# Autodesk Inventor assembly: 203.001.01_ZB_Modul
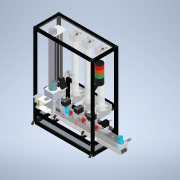
[picture p0: Inventor's stored thumbnail of the model, 180x180]
Saved by Autodesk Inventor 2022 (Build 260153000, 153)
## iProperties
Created: 2021-12-04
Part Number: 203.001.01_ZB_Modul
Document SubType Name: Assembly
Designer: Sebastian Seewald
Author: Sebastian Seewald
## Documents named in this file (18)
- C:\Users\kaebi\OneDrive - mci4me.at\03_MCI Master\4.Semester_SS2022\Masterarbeit\Software\CAD_TeachingFactory\203.001.01_ZB_Modul.iam
- C:\Users\kaebi\OneDrive - mci4me.at\03_MCI Master\4.Semester_SS2022\Masterarbeit\Software\CAD_TeachingFactory\202.002.01_ZB_Rahmen_Modul.iam
- C:\Users\kaebi\OneDrive - mci4me.at\03_MCI Master\4.Semester_SS2022\Masterarbeit\Software\CAD_TeachingFactory\503.001.01_Statuslampe.ipt
- C:\Users\kaebi\OneDrive - mci4me.at\03_MCI Master\4.Semester_SS2022\Masterarbeit\Software\CAD_TeachingFactory\DIN 934 - M4 x 0.7 Mutter.ipt
- C:\Users\kaebi\OneDrive - mci4me.at\03_MCI Master\4.Semester_SS2022\Masterarbeit\Software\CAD_TeachingFactory\204.006.01_ZB_Extrudereinheit.iam
- C:\Users\kaebi\OneDrive - mci4me.at\03_MCI Master\4.Semester_SS2022\Masterarbeit\Software\CAD_TeachingFactory\DIN 6902 - M4 Unterlegscheibe.ipt
- C:\Users\kaebi\OneDrive - mci4me.at\03_MCI Master\4.Semester_SS2022\Masterarbeit\Software\CAD_TeachingFactory\DIN 912 - M4 x 20.ipt
- C:\Users\kaebi\OneDrive - mci4me.at\03_MCI Master\4.Semester_SS2022\Masterarbeit\Software\CAD_TeachingFactory\204.005.01_ZB_Hubmagnetstopper.iam
- C:\Users\kaebi\OneDrive - mci4me.at\03_MCI Master\4.Semester_SS2022\Masterarbeit\Software\CAD_TeachingFactory\DIN EN ISO 4762 - M4 x 10.ipt
- C:\Users\kaebi\OneDrive - mci4me.at\03_MCI Master\4.Semester_SS2022\Masterarbeit\Software\CAD_TeachingFactory\205.001.01_ZB_Foerderbandeinheit.iam
- C:\Users\kaebi\OneDrive - mci4me.at\03_MCI Master\4.Semester_SS2022\Masterarbeit\Software\CAD_TeachingFactory\DIN_912_M3x8.ipt
- C:\Users\kaebi\OneDrive - mci4me.at\03_MCI Master\4.Semester_SS2022\Masterarbeit\Software\CAD_TeachingFactory\206.001.01_Vereinzelung_Gesamtbaugruppe.iam
- 206.001.01_Vereinzelung_Gesamtbaugruppe.iam
- C:\Users\kaebi\OneDrive - mci4me.at\03_MCI Master\4.Semester_SS2022\Masterarbeit\Software\CAD_TeachingFactory\503.002.01_Laborflaschen.ipt
- C:\Users\kaebi\OneDrive - mci4me.at\03_MCI Master\4.Semester_SS2022\Masterarbeit\Software\CAD_TeachingFactory\506.007.01_Linearaktor.iam
- C:\Users\kaebi\OneDrive - mci4me.at\03_MCI Master\4.Semester_SS2022\Masterarbeit\Software\CAD_TeachingFactory\106.023.01_Zapfen_Aktor.ipt
- C:\Users\kaebi\OneDrive - mci4me.at\03_MCI Master\4.Semester_SS2022\Masterarbeit\Software\CAD_TeachingFactory\106.024.01_Zapfen_Aktor_Auflage.ipt
- C:\Users\kaebi\OneDrive - mci4me.at\03_MCI Master\4.Semester_SS2022\Masterarbeit\Software\CAD_TeachingFactory\106.025.01_Anbindung_Aktor.ipt
## Components (70 placed, 16 different names)
1. 202.002.01_ZB_Rahmen_Modul:1 [sub-assembly] — Passend:1, Passend:2, Passend:3, Passend:6, Passend:7, Passend:8, Passend:9, Passend:10, Passend:11, Passend:12, Passend:13, Passend:14, Passend:15, Passend:16, Passend:17, Passend:18, Passend:19, Passend:20, Passend:21, Passend:22, Passend:23, Passend:24, Passend:25, Passend:26, Passend:27, Passend:28, Passend:65, Passend:66, Passend:67, Passend:68, Passend:69, Winkel:1, Winkel:2, Winkel:3, Passend:95, Fluchtend:1, Passend:96, Passend:121, Fluchtend:2, Passend:122, Passend:129, Passend:146, Fluchtend:5, Passend:147
2. 503.001.01_Statuslampe:1 — Passend:1, Passend:2, Passend:3, Passend:4, Passend:5
3. DIN 934 - M4 x 0.7 Mutter:1 — Passend:4, Passend:6
4. DIN 934 - M4 x 0.7 Mutter:2 — Passend:5, Passend:7
5. 204.006.01_ZB_Extrudereinheit:1 [sub-assembly] — Passend:8, Passend:13, Passend:14, Passend:29, Passend:30, Passend:31, Passend:32, Passend:97, Passend:98, Passend:128
6. 204.006.01_ZB_Extrudereinheit:2 [sub-assembly] — Passend:9, Passend:12, Passend:15, Passend:33, Passend:34, Passend:35, Passend:36, Passend:99, Passend:100, Passend:127
7. 204.006.01_ZB_Extrudereinheit:3 [sub-assembly] — Passend:10, Passend:11, Passend:16, Passend:37, Passend:38, Passend:39, Passend:40, Passend:101, Passend:102, Passend:124, Fluchtend:3
8. DIN 6902 - M4 Unterlegscheibe:1 — Passend:20, Passend:37, Passend:43, Passend:55
9. DIN 6902 - M4 Unterlegscheibe:2 — Passend:18, Passend:39, Passend:41, Passend:53
10. DIN 6902 - M4 Unterlegscheibe:3 — Passend:17, Passend:40, Passend:42, Passend:54
11. DIN 6902 - M4 Unterlegscheibe:4 — Passend:19, Passend:38, Passend:44, Passend:56
12. DIN 6902 - M4 Unterlegscheibe:5 — Passend:21, Passend:36, Passend:46, Passend:58
13. DIN 6902 - M4 Unterlegscheibe:6 — Passend:23, Passend:34, Passend:48, Passend:60
14. DIN 6902 - M4 Unterlegscheibe:7 — Passend:22, Passend:35, Passend:45, Passend:57
15. DIN 6902 - M4 Unterlegscheibe:8 — Passend:25, Passend:30, Passend:52, Passend:63
16. DIN 6902 - M4 Unterlegscheibe:9 — Passend:26, Passend:31, Passend:51, Passend:61
17. DIN 6902 - M4 Unterlegscheibe:10 — Passend:24, Passend:33, Passend:47, Passend:59
18. DIN 6902 - M4 Unterlegscheibe:11 — Passend:28, Passend:29, Passend:50, Passend:64
19. DIN 6902 - M4 Unterlegscheibe:12 — Passend:27, Passend:32, Passend:49, Passend:62
20. DIN 912 - M4 x 20:1 — Passend:41, Passend:53
21. DIN 912 - M4 x 20:2 — Passend:44, Passend:56
22. DIN 912 - M4 x 20:3 — Passend:48, Passend:60
23. DIN 912 - M4 x 20:4 — Passend:51, Passend:61
24. DIN 912 - M4 x 20:5 — Passend:52, Passend:63
25. DIN 912 - M4 x 20:6 — Passend:47, Passend:59
26. DIN 912 - M4 x 20:7 — Passend:46, Passend:58
27. DIN 912 - M4 x 20:8 — Passend:43, Passend:55
28. DIN 912 - M4 x 20:9 — Passend:42, Passend:54
29. DIN 912 - M4 x 20:10 — Passend:45, Passend:57
30. DIN 912 - M4 x 20:11 — Passend:49, Passend:62
31. DIN 912 - M4 x 20:12 — Passend:50, Passend:64
32. 204.005.01_ZB_Hubmagnetstopper:1 [sub-assembly] — Passend:66, Passend:69, Winkel:2, Passend:76, Passend:77, Passend:78, Passend:79, Passend:85, Passend:86, Passend:91, Passend:92, Passend:127
33. 204.005.01_ZB_Hubmagnetstopper:2 [sub-assembly] — Passend:65, Winkel:1, Passend:80, Passend:81, Passend:82, Passend:83, Passend:87, Passend:88, Passend:89, Passend:90, Fluchtend:3
34. 204.005.01_ZB_Hubmagnetstopper:3 [sub-assembly] — Passend:67, Passend:68, Winkel:3, Passend:71, Passend:72, Passend:73, Passend:74, Passend:75, Passend:84, Passend:93, Passend:94, Passend:128
35. DIN EN ISO 4762 - M4 x 10:1 — Passend:71, Passend:72
36. DIN EN ISO 4762 - M4 x 10:2 — Passend:75, Passend:93
37. DIN EN ISO 4762 - M4 x 10:3 — Passend:74, Passend:94
38. DIN EN ISO 4762 - M4 x 10:4 — Passend:73, Passend:84
39. DIN EN ISO 4762 - M4 x 10:5 — Passend:76, Passend:85
40. DIN EN ISO 4762 - M4 x 10:6 — Passend:77, Passend:92
41. DIN EN ISO 4762 - M4 x 10:7 — Passend:78, Passend:86
42. DIN EN ISO 4762 - M4 x 10:8 — Passend:79, Passend:91
43. DIN EN ISO 4762 - M4 x 10:9 — Passend:82, Passend:90
44. DIN EN ISO 4762 - M4 x 10:10 — Passend:83, Passend:89
45. DIN EN ISO 4762 - M4 x 10:11 — Passend:81, Passend:88
46. DIN EN ISO 4762 - M4 x 10:12 — Passend:80, Passend:87, Passend:129
47. 205.001.01_ZB_Foerderbandeinheit:1 [sub-assembly] — Passend:95, Fluchtend:1, Passend:96, Passend:103, Passend:104, Passend:105, Passend:106, Passend:107, Passend:108, Passend:115, Passend:116, Passend:117, Passend:118, Passend:119, Passend:120, Passend:123, Passend:125, Passend:130, Passend:131
48. DIN_912_M3x8:1 — Passend:97, Passend:103, Passend:109
49. DIN_912_M3x8:2 — Passend:98, Passend:104, Passend:110
50. DIN_912_M3x8:3 — Passend:99, Passend:105, Passend:111
51. DIN_912_M3x8:4 — Passend:100, Passend:106, Passend:112
52. DIN_912_M3x8:5 — Passend:102, Passend:108, Passend:114
53. DIN_912_M3x8:6 — Passend:101, Passend:107, Passend:113
54. DIN_912_M3x8:7 — Passend:110, Passend:119
55. DIN_912_M3x8:8 — Passend:109, Passend:120
56. DIN_912_M3x8:9 — Passend:112, Passend:117
57. DIN_912_M3x8:10 — Passend:111, Passend:118
58. DIN_912_M3x8:11 — Passend:113, Passend:116
59. DIN_912_M3x8:12 — Passend:114, Passend:115
60. 206.001.01_Vereinzelung_Gesamtbaugruppe:1 [sub-assembly] — Passend:121, Fluchtend:2, Passend:122, Passend:148, Passend:149
61. 503.002.01_Laborflaschen:1 — Passend:123, Passend:124, Passend:125
62. 503.002.01_Laborflaschen:2 — Passend:130, Passend:131
63. 506.007.01_Linearaktor:1 [sub-assembly] — Passend:148
64. 102.004.01_Zapfen_Aktor:1
65. 102.004.01_Zapfen_Aktor:2
66. 102.005.01_Zapfen_Aktor_Auflage:1
67. 102.005.01_Zapfen_Aktor_Auflage:2
68. 106.025.01_Anbindung_Aktor:1
69. 106.025.01_Anbindung_Aktor:2 — Passend:146, Fluchtend:5, Passend:147
70. 506.007.01_Linearaktor:2 [sub-assembly] — Passend:149
## Relationships (155: Mate 147, Flush 5, Angle 3)
- Passend:1 [Mate]: 202.002.01_ZB_Rahmen_Modul:1 ↔ 503.001.01_Statuslampe:1
- Passend:2 [Mate]: 202.002.01_ZB_Rahmen_Modul:1 ↔ 503.001.01_Statuslampe:1
- Passend:3 [Mate]: 202.002.01_ZB_Rahmen_Modul:1 ↔ 503.001.01_Statuslampe:1
- Passend:4 [Mate]: 503.001.01_Statuslampe:1 ↔ DIN 934 - M4 x 0.7 Mutter:1
- Passend:5 [Mate]: 503.001.01_Statuslampe:1 ↔ DIN 934 - M4 x 0.7 Mutter:2
- Passend:6 [Mate]: 202.002.01_ZB_Rahmen_Modul:1 ↔ DIN 934 - M4 x 0.7 Mutter:1
- Passend:7 [Mate]: 202.002.01_ZB_Rahmen_Modul:1 ↔ DIN 934 - M4 x 0.7 Mutter:2
- Passend:8 [Mate]: 202.002.01_ZB_Rahmen_Modul:1 ↔ 204.006.01_ZB_Extrudereinheit:1
- Passend:9 [Mate]: 202.002.01_ZB_Rahmen_Modul:1 ↔ 204.006.01_ZB_Extrudereinheit:2
- Passend:10 [Mate]: 202.002.01_ZB_Rahmen_Modul:1 ↔ 204.006.01_ZB_Extrudereinheit:3
- Passend:11 [Mate] (-10 mm): 202.002.01_ZB_Rahmen_Modul:1 ↔ 204.006.01_ZB_Extrudereinheit:3
- Passend:12 [Mate] (-10 mm): 202.002.01_ZB_Rahmen_Modul:1 ↔ 204.006.01_ZB_Extrudereinheit:2
- Passend:13 [Mate] (-10 mm): 202.002.01_ZB_Rahmen_Modul:1 ↔ 204.006.01_ZB_Extrudereinheit:1
- Passend:14 [Mate]: 202.002.01_ZB_Rahmen_Modul:1 ↔ 204.006.01_ZB_Extrudereinheit:1
- Passend:15 [Mate]: 202.002.01_ZB_Rahmen_Modul:1 ↔ 204.006.01_ZB_Extrudereinheit:2
- Passend:16 [Mate]: 202.002.01_ZB_Rahmen_Modul:1 ↔ 204.006.01_ZB_Extrudereinheit:3
- Passend:17 [Mate]: 202.002.01_ZB_Rahmen_Modul:1 ↔ DIN 6902 - M4 Unterlegscheibe:3
- Passend:18 [Mate]: 202.002.01_ZB_Rahmen_Modul:1 ↔ DIN 6902 - M4 Unterlegscheibe:2
- Passend:19 [Mate]: 202.002.01_ZB_Rahmen_Modul:1 ↔ DIN 6902 - M4 Unterlegscheibe:4
- Passend:20 [Mate]: 202.002.01_ZB_Rahmen_Modul:1 ↔ DIN 6902 - M4 Unterlegscheibe:1
- Passend:21 [Mate]: 202.002.01_ZB_Rahmen_Modul:1 ↔ DIN 6902 - M4 Unterlegscheibe:5
- Passend:22 [Mate]: 202.002.01_ZB_Rahmen_Modul:1 ↔ DIN 6902 - M4 Unterlegscheibe:7
- Passend:23 [Mate]: 202.002.01_ZB_Rahmen_Modul:1 ↔ DIN 6902 - M4 Unterlegscheibe:6
- Passend:24 [Mate]: 202.002.01_ZB_Rahmen_Modul:1 ↔ DIN 6902 - M4 Unterlegscheibe:10
- Passend:25 [Mate]: 202.002.01_ZB_Rahmen_Modul:1 ↔ DIN 6902 - M4 Unterlegscheibe:8
- Passend:26 [Mate]: 202.002.01_ZB_Rahmen_Modul:1 ↔ DIN 6902 - M4 Unterlegscheibe:9
- Passend:27 [Mate]: 202.002.01_ZB_Rahmen_Modul:1 ↔ DIN 6902 - M4 Unterlegscheibe:12
- Passend:28 [Mate]: 202.002.01_ZB_Rahmen_Modul:1 ↔ DIN 6902 - M4 Unterlegscheibe:11
- Passend:29 [Mate]: 204.006.01_ZB_Extrudereinheit:1 ↔ DIN 6902 - M4 Unterlegscheibe:11
- Passend:30 [Mate]: 204.006.01_ZB_Extrudereinheit:1 ↔ DIN 6902 - M4 Unterlegscheibe:8
- Passend:31 [Mate]: 204.006.01_ZB_Extrudereinheit:1 ↔ DIN 6902 - M4 Unterlegscheibe:9
- Passend:32 [Mate]: 204.006.01_ZB_Extrudereinheit:1 ↔ DIN 6902 - M4 Unterlegscheibe:12
- Passend:33 [Mate]: 204.006.01_ZB_Extrudereinheit:2 ↔ DIN 6902 - M4 Unterlegscheibe:10
- Passend:34 [Mate]: 204.006.01_ZB_Extrudereinheit:2 ↔ DIN 6902 - M4 Unterlegscheibe:6
- Passend:35 [Mate]: 204.006.01_ZB_Extrudereinheit:2 ↔ DIN 6902 - M4 Unterlegscheibe:7
- Passend:36 [Mate]: 204.006.01_ZB_Extrudereinheit:2 ↔ DIN 6902 - M4 Unterlegscheibe:5
- Passend:37 [Mate]: 204.006.01_ZB_Extrudereinheit:3 ↔ DIN 6902 - M4 Unterlegscheibe:1
- Passend:38 [Mate]: 204.006.01_ZB_Extrudereinheit:3 ↔ DIN 6902 - M4 Unterlegscheibe:4
- Passend:39 [Mate]: 204.006.01_ZB_Extrudereinheit:3 ↔ DIN 6902 - M4 Unterlegscheibe:2
- Passend:40 [Mate]: 204.006.01_ZB_Extrudereinheit:3 ↔ DIN 6902 - M4 Unterlegscheibe:3
- Passend:41 [Mate]: DIN 6902 - M4 Unterlegscheibe:2 ↔ DIN 912 - M4 x 20:1
- Passend:42 [Mate]: DIN 6902 - M4 Unterlegscheibe:3 ↔ DIN 912 - M4 x 20:9
- Passend:43 [Mate]: DIN 6902 - M4 Unterlegscheibe:1 ↔ DIN 912 - M4 x 20:8
- Passend:44 [Mate]: DIN 6902 - M4 Unterlegscheibe:4 ↔ DIN 912 - M4 x 20:2
- Passend:45 [Mate]: DIN 6902 - M4 Unterlegscheibe:7 ↔ DIN 912 - M4 x 20:10
- Passend:46 [Mate]: DIN 6902 - M4 Unterlegscheibe:5 ↔ DIN 912 - M4 x 20:7
- Passend:47 [Mate]: DIN 6902 - M4 Unterlegscheibe:10 ↔ DIN 912 - M4 x 20:6
- Passend:48 [Mate]: DIN 6902 - M4 Unterlegscheibe:6 ↔ DIN 912 - M4 x 20:3
- Passend:49 [Mate]: DIN 6902 - M4 Unterlegscheibe:12 ↔ DIN 912 - M4 x 20:11
- Passend:50 [Mate]: DIN 6902 - M4 Unterlegscheibe:11 ↔ DIN 912 - M4 x 20:12
- Passend:51 [Mate]: DIN 6902 - M4 Unterlegscheibe:9 ↔ DIN 912 - M4 x 20:4
- Passend:52 [Mate]: DIN 6902 - M4 Unterlegscheibe:8 ↔ DIN 912 - M4 x 20:5
- Passend:53 [Mate]: DIN 6902 - M4 Unterlegscheibe:2 ↔ DIN 912 - M4 x 20:1
- Passend:54 [Mate]: DIN 6902 - M4 Unterlegscheibe:3 ↔ DIN 912 - M4 x 20:9
- Passend:55 [Mate]: DIN 6902 - M4 Unterlegscheibe:1 ↔ DIN 912 - M4 x 20:8
- Passend:56 [Mate]: DIN 6902 - M4 Unterlegscheibe:4 ↔ DIN 912 - M4 x 20:2
- Passend:57 [Mate]: DIN 6902 - M4 Unterlegscheibe:7 ↔ DIN 912 - M4 x 20:10
- Passend:58 [Mate]: DIN 6902 - M4 Unterlegscheibe:5 ↔ DIN 912 - M4 x 20:7
- Passend:59 [Mate]: DIN 6902 - M4 Unterlegscheibe:10 ↔ DIN 912 - M4 x 20:6
- Passend:60 [Mate]: DIN 6902 - M4 Unterlegscheibe:6 ↔ DIN 912 - M4 x 20:3
- Passend:61 [Mate]: DIN 6902 - M4 Unterlegscheibe:9 ↔ DIN 912 - M4 x 20:4
- Passend:62 [Mate]: DIN 6902 - M4 Unterlegscheibe:12 ↔ DIN 912 - M4 x 20:11
- Passend:63 [Mate]: DIN 6902 - M4 Unterlegscheibe:8 ↔ DIN 912 - M4 x 20:5
- Passend:64 [Mate]: DIN 6902 - M4 Unterlegscheibe:11 ↔ DIN 912 - M4 x 20:12
- Passend:65 [Mate]: 202.002.01_ZB_Rahmen_Modul:1 ↔ 204.005.01_ZB_Hubmagnetstopper:2
- Passend:66 [Mate]: 202.002.01_ZB_Rahmen_Modul:1 ↔ 204.005.01_ZB_Hubmagnetstopper:1
- Passend:67 [Mate]: 202.002.01_ZB_Rahmen_Modul:1 ↔ 204.005.01_ZB_Hubmagnetstopper:3
- Passend:68 [Mate] (-10 mm): 202.002.01_ZB_Rahmen_Modul:1 ↔ 204.005.01_ZB_Hubmagnetstopper:3
- Passend:69 [Mate] (-10 mm): 202.002.01_ZB_Rahmen_Modul:1 ↔ 204.005.01_ZB_Hubmagnetstopper:1
- Winkel:1 [Angle] (0 deg): 202.002.01_ZB_Rahmen_Modul:1 ↔ 204.005.01_ZB_Hubmagnetstopper:2
- Winkel:2 [Angle] (0 deg): 202.002.01_ZB_Rahmen_Modul:1 ↔ 204.005.01_ZB_Hubmagnetstopper:1
- Winkel:3 [Angle] (0 deg): 202.002.01_ZB_Rahmen_Modul:1 ↔ 204.005.01_ZB_Hubmagnetstopper:3
- Passend:71 [Mate]: 204.005.01_ZB_Hubmagnetstopper:3 ↔ DIN EN ISO 4762 - M4 x 10:1
- Passend:72 [Mate]: 204.005.01_ZB_Hubmagnetstopper:3 ↔ DIN EN ISO 4762 - M4 x 10:1
- Passend:73 [Mate]: 204.005.01_ZB_Hubmagnetstopper:3 ↔ DIN EN ISO 4762 - M4 x 10:4
- Passend:74 [Mate]: 204.005.01_ZB_Hubmagnetstopper:3 ↔ DIN EN ISO 4762 - M4 x 10:3
- Passend:75 [Mate]: 204.005.01_ZB_Hubmagnetstopper:3 ↔ DIN EN ISO 4762 - M4 x 10:2
- Passend:76 [Mate]: 204.005.01_ZB_Hubmagnetstopper:1 ↔ DIN EN ISO 4762 - M4 x 10:5
- Passend:77 [Mate]: 204.005.01_ZB_Hubmagnetstopper:1 ↔ DIN EN ISO 4762 - M4 x 10:6
- Passend:78 [Mate]: 204.005.01_ZB_Hubmagnetstopper:1 ↔ DIN EN ISO 4762 - M4 x 10:7
- Passend:79 [Mate]: 204.005.01_ZB_Hubmagnetstopper:1 ↔ DIN EN ISO 4762 - M4 x 10:8
- Passend:80 [Mate]: 204.005.01_ZB_Hubmagnetstopper:2 ↔ DIN EN ISO 4762 - M4 x 10:12
- Passend:81 [Mate]: 204.005.01_ZB_Hubmagnetstopper:2 ↔ DIN EN ISO 4762 - M4 x 10:11
- Passend:82 [Mate]: 204.005.01_ZB_Hubmagnetstopper:2 ↔ DIN EN ISO 4762 - M4 x 10:9
- Passend:83 [Mate]: 204.005.01_ZB_Hubmagnetstopper:2 ↔ DIN EN ISO 4762 - M4 x 10:10
- Passend:84 [Mate]: 204.005.01_ZB_Hubmagnetstopper:3 ↔ DIN EN ISO 4762 - M4 x 10:4
- Passend:85 [Mate]: 204.005.01_ZB_Hubmagnetstopper:1 ↔ DIN EN ISO 4762 - M4 x 10:5
- Passend:86 [Mate]: 204.005.01_ZB_Hubmagnetstopper:1 ↔ DIN EN ISO 4762 - M4 x 10:7
- Passend:87 [Mate]: 204.005.01_ZB_Hubmagnetstopper:2 ↔ DIN EN ISO 4762 - M4 x 10:12
- Passend:88 [Mate]: 204.005.01_ZB_Hubmagnetstopper:2 ↔ DIN EN ISO 4762 - M4 x 10:11
- Passend:89 [Mate]: 204.005.01_ZB_Hubmagnetstopper:2 ↔ DIN EN ISO 4762 - M4 x 10:10
- Passend:90 [Mate]: 204.005.01_ZB_Hubmagnetstopper:2 ↔ DIN EN ISO 4762 - M4 x 10:9
- Passend:91 [Mate]: 204.005.01_ZB_Hubmagnetstopper:1 ↔ DIN EN ISO 4762 - M4 x 10:8
- Passend:92 [Mate]: 204.005.01_ZB_Hubmagnetstopper:1 ↔ DIN EN ISO 4762 - M4 x 10:6
- Passend:93 [Mate]: 204.005.01_ZB_Hubmagnetstopper:3 ↔ DIN EN ISO 4762 - M4 x 10:2
- Passend:94 [Mate]: 204.005.01_ZB_Hubmagnetstopper:3 ↔ DIN EN ISO 4762 - M4 x 10:3
- Passend:95 [Mate]: 202.002.01_ZB_Rahmen_Modul:1 ↔ 205.001.01_ZB_Foerderbandeinheit:1
- Fluchtend:1 [Flush]: 202.002.01_ZB_Rahmen_Modul:1 ↔ 205.001.01_ZB_Foerderbandeinheit:1
- Passend:96 [Mate] (5 mm): 202.002.01_ZB_Rahmen_Modul:1 ↔ 205.001.01_ZB_Foerderbandeinheit:1
- Passend:97 [Mate]: 204.006.01_ZB_Extrudereinheit:1 ↔ DIN_912_M3x8:1
- Passend:98 [Mate]: 204.006.01_ZB_Extrudereinheit:1 ↔ DIN_912_M3x8:2
- Passend:99 [Mate]: 204.006.01_ZB_Extrudereinheit:2 ↔ DIN_912_M3x8:3
- Passend:100 [Mate]: 204.006.01_ZB_Extrudereinheit:2 ↔ DIN_912_M3x8:4
- Passend:101 [Mate]: 204.006.01_ZB_Extrudereinheit:3 ↔ DIN_912_M3x8:6
- Passend:102 [Mate]: 204.006.01_ZB_Extrudereinheit:3 ↔ DIN_912_M3x8:5
- Passend:103 [Mate]: 205.001.01_ZB_Foerderbandeinheit:1 ↔ DIN_912_M3x8:1
- Passend:104 [Mate]: 205.001.01_ZB_Foerderbandeinheit:1 ↔ DIN_912_M3x8:2
- Passend:105 [Mate]: 205.001.01_ZB_Foerderbandeinheit:1 ↔ DIN_912_M3x8:3
- Passend:106 [Mate]: 205.001.01_ZB_Foerderbandeinheit:1 ↔ DIN_912_M3x8:4
- Passend:107 [Mate]: 205.001.01_ZB_Foerderbandeinheit:1 ↔ DIN_912_M3x8:6
- Passend:108 [Mate]: 205.001.01_ZB_Foerderbandeinheit:1 ↔ DIN_912_M3x8:5
- Passend:109 [Mate]: DIN_912_M3x8:1 ↔ DIN_912_M3x8:8
- Passend:110 [Mate]: DIN_912_M3x8:2 ↔ DIN_912_M3x8:7
- Passend:111 [Mate]: DIN_912_M3x8:3 ↔ DIN_912_M3x8:10
- Passend:112 [Mate]: DIN_912_M3x8:4 ↔ DIN_912_M3x8:9
- Passend:113 [Mate]: DIN_912_M3x8:6 ↔ DIN_912_M3x8:11
- Passend:114 [Mate]: DIN_912_M3x8:5 ↔ DIN_912_M3x8:12
- Passend:115 [Mate]: 205.001.01_ZB_Foerderbandeinheit:1 ↔ DIN_912_M3x8:12
- Passend:116 [Mate]: 205.001.01_ZB_Foerderbandeinheit:1 ↔ DIN_912_M3x8:11
- Passend:117 [Mate]: 205.001.01_ZB_Foerderbandeinheit:1 ↔ DIN_912_M3x8:9
- Passend:118 [Mate]: 205.001.01_ZB_Foerderbandeinheit:1 ↔ DIN_912_M3x8:10
- Passend:119 [Mate]: 205.001.01_ZB_Foerderbandeinheit:1 ↔ DIN_912_M3x8:7
- Passend:120 [Mate]: 205.001.01_ZB_Foerderbandeinheit:1 ↔ DIN_912_M3x8:8
- Passend:121 [Mate]: 202.002.01_ZB_Rahmen_Modul:1 ↔ 206.001.01_Vereinzelung_Gesamtbaugruppe:1
- Fluchtend:2 [Flush]: 202.002.01_ZB_Rahmen_Modul:1 ↔ 206.001.01_Vereinzelung_Gesamtbaugruppe:1
- Passend:122 [Mate]: 202.002.01_ZB_Rahmen_Modul:1 ↔ 206.001.01_Vereinzelung_Gesamtbaugruppe:1
- Passend:123 [Mate]: 205.001.01_ZB_Foerderbandeinheit:1 ↔ 503.002.01_Laborflaschen:1
- Passend:124 [Mate] (-17.5 mm): 204.006.01_ZB_Extrudereinheit:3 ↔ 503.002.01_Laborflaschen:1
- Passend:125 [Mate] (-30 mm): 205.001.01_ZB_Foerderbandeinheit:1 ↔ 503.002.01_Laborflaschen:1
- Passend:127 [Mate] (-17.5 mm): 204.006.01_ZB_Extrudereinheit:2 ↔ 204.005.01_ZB_Hubmagnetstopper:1
- Passend:128 [Mate] (-17.5 mm): 204.006.01_ZB_Extrudereinheit:1 ↔ 204.005.01_ZB_Hubmagnetstopper:3
- Passend:129 [Mate] (-10 mm): 202.002.01_ZB_Rahmen_Modul:1 ↔ DIN EN ISO 4762 - M4 x 10:12
- Fluchtend:3 [Flush] (-4 mm): 204.006.01_ZB_Extrudereinheit:3 ↔ 204.005.01_ZB_Hubmagnetstopper:2
- Passend:130 [Mate]: 205.001.01_ZB_Foerderbandeinheit:1 ↔ 503.002.01_Laborflaschen:2
- Passend:131 [Mate]: 205.001.01_ZB_Foerderbandeinheit:1 ↔ 503.002.01_Laborflaschen:2
- [Mate] (1 mm): 506.007.01_Linearaktor:1 ↔ 102.004.01_Zapfen_Aktor:2
- [Mate]: 506.007.01_Linearaktor:1 ↔ 102.004.01_Zapfen_Aktor:2
- [Mate]: 102.004.01_Zapfen_Aktor:2 ↔ 102.005.01_Zapfen_Aktor_Auflage:2
- [Mate]: 102.004.01_Zapfen_Aktor:2 ↔ 102.005.01_Zapfen_Aktor_Auflage:2
- [Mate]: 102.004.01_Zapfen_Aktor:1 ↔ 102.005.01_Zapfen_Aktor_Auflage:1
- [Mate]: 102.004.01_Zapfen_Aktor:1 ↔ 102.005.01_Zapfen_Aktor_Auflage:1
- [Mate]: 102.005.01_Zapfen_Aktor_Auflage:2 ↔ 106.025.01_Anbindung_Aktor:2
- [Mate]: 102.005.01_Zapfen_Aktor_Auflage:1 ↔ 106.025.01_Anbindung_Aktor:2
- [Mate]: 102.005.01_Zapfen_Aktor_Auflage:2 ↔ 106.025.01_Anbindung_Aktor:2
- [Mate]: 102.004.01_Zapfen_Aktor:1 ↔ 506.007.01_Linearaktor:2
- [Mate] (1 mm): 102.004.01_Zapfen_Aktor:1 ↔ 506.007.01_Linearaktor:2
- [Flush]: 506.007.01_Linearaktor:1 ↔ 506.007.01_Linearaktor:2
- [Mate]: 102.004.01_Zapfen_Aktor:1 ↔ 106.025.01_Anbindung_Aktor:1
- [Mate]: 102.004.01_Zapfen_Aktor:2 ↔ 106.025.01_Anbindung_Aktor:1
- [Mate]: 102.004.01_Zapfen_Aktor:2 ↔ 106.025.01_Anbindung_Aktor:1
- Passend:146 [Mate]: 202.002.01_ZB_Rahmen_Modul:1 ↔ 106.025.01_Anbindung_Aktor:2
- Fluchtend:5 [Flush]: 202.002.01_ZB_Rahmen_Modul:1 ↔ 106.025.01_Anbindung_Aktor:2
- Passend:147 [Mate]: 202.002.01_ZB_Rahmen_Modul:1 ↔ 106.025.01_Anbindung_Aktor:2
- Passend:148 [Mate]: 206.001.01_Vereinzelung_Gesamtbaugruppe:1 ↔ 506.007.01_Linearaktor:1
- Passend:149 [Mate]: 206.001.01_Vereinzelung_Gesamtbaugruppe:1 ↔ 506.007.01_Linearaktor:2
## Named parameters: d139_d81 = 0 mm, d140_d82 = 0 mm, d141_d83 = 0 mm, d142_d77 = 0 mm, d143_d78 = 1 mm, d144_d79 = 0 mm, d145_d0 = 1 mm, d146_d1 = 0 mm, d147_d4 = 0 mm, d148_d5 = 0 mm, d149_d6 = 0 mm, d150_d7 = 0 mm, d11_d6 = 0 mm, d12_d7 = 0 mm, d153_d8 = 0 mm
